# Autodesk Inventor assembly: AN929-10D
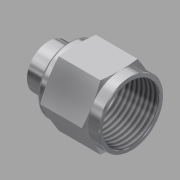
[picture p0: Inventor's stored thumbnail of the model, 180x180]
Saved by Autodesk Inventor 2019 (Build 230136000, 136)
## iProperties
Created: 2018-11-23
Part Number: AN929-10D
Document SubType Name: Assembly
Designer: erics
Mass: 23.2538 g
Surface Area: 61.5994 cm^2
Volume: 8.33688 cm^3
Density: 2.78927 g/cm^3
Author: erics
## Documents named in this file (6)
- D:\Users\erics\Documents\CAD Library\Pipe Fittings\AN-MS-Fittings\AN929\AN929-10D.iam
- D:\Users\erics\Documents\CAD Library\Pipe Fittings\AN-MS-Fittings\AN929.ipt
- D:\Users\erics\Documents\CAD Library\Pipe Fittings\AN-MS-Fittings\AN818.ipt
- D:\Users\erics\Documents\CAD Library\Pipe Fittings\AN-MS-Fittings\AN929.iam
- D:\Users\erics\Documents\CAD Library\Pipe Fittings\AN-MS-Fittings\AN929\AN929-10D.ipt
- D:\Users\erics\Documents\CAD Library\Pipe Fittings\AN-MS-Fittings\AN818\AN818-10D.ipt
## Components (2 placed, 2 different names)
1. AN929-10D:1 — Insert:1
2. AN818-10D:1 — Insert:1
## Relationships (1: Insert 1)
- Insert:1: AN929-10D:1 ↔ AN818-10D:1
